# Autodesk Inventor assembly: Assembly1
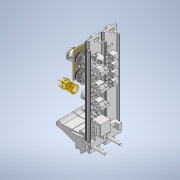
[picture p0: Inventor's stored thumbnail of the model, 180x180]
Saved by Autodesk Inventor 2022 (Build 260153000, 153)
## iProperties
Created: 2021-06-11
Part Number: Assembly1
Document SubType Name: Assembly
Designer: capta
Author: capta
## Documents named in this file (9)
- C:\Users\capta\OneDrive - Lehigh University\Research\High-Speed ML\pxi_impedance_pcb_cad\Assembly1.iam
- C:\Users\capta\OneDrive - Lehigh University\Research\High-Speed ML\pxi_impedance_pcb_cad\cu_pxi-5412.ipt
- C:\Users\capta\OneDrive - Lehigh University\Research\High-Speed ML\pxi_impedance_pcb_cad\cu_pxie-1085.ipt
- C:\Users\capta\OneDrive - Lehigh University\Research\High-Speed ML\pxi_impedance_pcb_cad\cu_pxie-5122.ipt
- C:\Users\capta\Desktop\BNC Connector (Male).ipt
- C:\Users\capta\Downloads\CONSMB006-G--3DModel-STEP-56544.ipt
- C:\Users\capta\Downloads\impedance_measure1(5).ipt
- C:\Users\capta\OneDrive - Lehigh University\Research\High-Speed ML\pxi_impedance_pcb_cad\spacer1.ipt
- C:\Users\capta\Desktop\112404.ipt
## Components (9 placed, 8 different names)
1. cu_pxi-5412:1 — Mate:1, Angle:1, Mate:2, Flush:1, Angle:2
2. cu_pxie-1085:1 — Mate:1, Angle:1, Mate:2, Mate:3
3. cu_pxie-5122:1 — Flush:1, Mate:3, Angle:2, Mate:4, Mate:5
4. BNC Connector (Male):1
5. CONSMB006-G--3DModel-STEP-56544:1
6. impedance_measure1(5):1 — Mate:4, Mate:5, Mate:6, Mate:7, Mate:9
7. spacer1:1 — Mate:6, Mate:7, Mate:8
8. CONSMB006-G--3DModel-STEP-56544:2 — Mate:8, Mate:9
9. 112404:1
## Relationships (12: Mate 9, Angle 2, Flush 1)
- Mate:1: cu_pxi-5412:1 ↔ cu_pxie-1085:1
- Angle:1 (0 deg): cu_pxi-5412:1 ↔ cu_pxie-1085:1
- Mate:2: cu_pxi-5412:1 ↔ cu_pxie-1085:1
- Flush:1: cu_pxi-5412:1 ↔ cu_pxie-5122:1
- Mate:3: cu_pxie-1085:1 ↔ cu_pxie-5122:1
- Angle:2 (0 deg): cu_pxi-5412:1 ↔ cu_pxie-5122:1
- Mate:4: cu_pxie-5122:1 ↔ impedance_measure1(5):1
- Mate:5: cu_pxie-5122:1 ↔ impedance_measure1(5):1
- Mate:6: impedance_measure1(5):1 ↔ spacer1:1
- Mate:7: impedance_measure1(5):1 ↔ spacer1:1
- Mate:8: spacer1:1 ↔ CONSMB006-G--3DModel-STEP-56544:2
- Mate:9: impedance_measure1(5):1 ↔ CONSMB006-G--3DModel-STEP-56544:2
